# Autodesk Inventor assembly: servoribbon
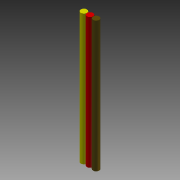
[picture p0: Inventor's stored thumbnail of the model, 180x180]
Saved by Autodesk Inventor 2012 (Build 160160000, 160)
## iProperties
Created: 2014-07-18
Part Number: servoribbon
Document SubType Name: Assembly
Designer: Anon
Author: Anon
## Documents named in this file (4)
- D:\Dropbox\Courses\GP\git\dronestructure\electronics\afroesc\servoribbon.iam
- D:\Dropbox\Courses\GP\git\dronestructure\electronics\afroesc\brownribbon.ipt
- D:\Dropbox\Courses\GP\git\dronestructure\electronics\afroesc\redribbon.ipt
- D:\Dropbox\Courses\GP\git\dronestructure\electronics\afroesc\yellowribbon.ipt
## Components (3 placed, 3 different names)
1. brownribbon:1 — Flush:1, Flush:2, Tangent:1, Flush:3
2. redribbon:1 — Flush:1, Tangent:1, Tangent:2, Mate:1, Mate:2
3. yellowribbon:1 — Flush:2, Tangent:2, Mate:2
## Relationships (7: Flush 3, Tangent 2, Mate 2)
- Flush:1: brownribbon:1 ↔ redribbon:1
- Flush:2: brownribbon:1 ↔ yellowribbon:1
- Tangent:1: brownribbon:1 ↔ redribbon:1
- Tangent:2: redribbon:1 ↔ yellowribbon:1
- Flush:3: brownribbon:1
- Mate:1: redribbon:1
- Mate:2: redribbon:1 ↔ yellowribbon:1
